# Autodesk Inventor assembly: soportes
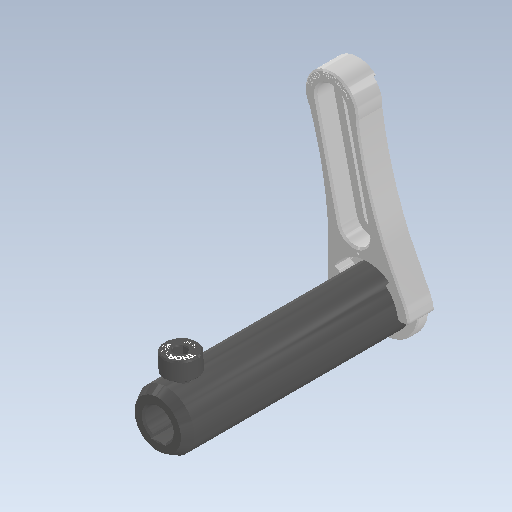
[picture p0: Inventor's stored thumbnail of the model, 512x512]
Saved by Autodesk Inventor 2020 (Build 240168000, 168)
## iProperties
Created: 2022-10-17
Part Number: soportes
Document SubType Name: Assembly
Designer: General
Author: General
## Documents named in this file (3)
- C:\LAFriOC\diseños\sistema de vacío\soportes.iam
- C:\LAFriOC\diseños\sistema de vacío\PH100E_M-Solidworks.ipt
- C:\LAFriOC\diseños\sistema de vacío\CF175-Solidworks.ipt
## Components (2 placed, 2 different names)
1. PH100E_M-Solidworks:1 — Insertar:1
2. CF175-Solidworks:1 — Insertar:1
## Relationships (1: Insert 1)
- Insertar:1: PH100E_M-Solidworks:1 ↔ CF175-Solidworks:1
